# Autodesk Inventor assembly: Motor Panel
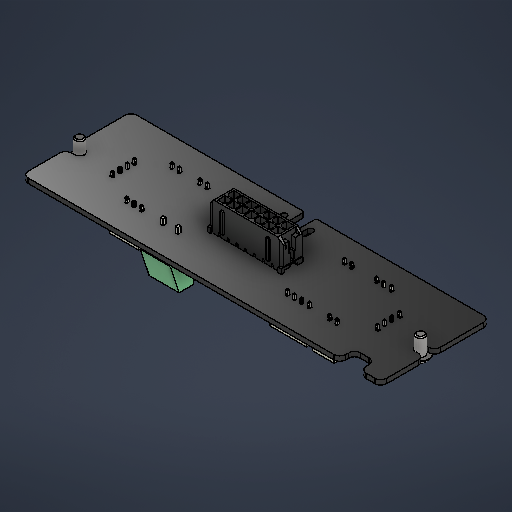
[picture p0: Inventor's stored thumbnail of the model, 512x512]
Saved by Autodesk Inventor 2026.1 (Build 301233020, 233B)
## iProperties
Created: 2025-05-09
Part Number: Motor Panel
Document SubType Name: Assembly
Designer: AdminForWorker
Title: Motor Panel
Author: AdminForWorker
## Documents named in this file (8)
- C:\Users\JoshuaEah\Documents\GitHub\Voron-0\CAD\Master Assembly\Panels\Subassemblies\Motor Panel.iam
- C:\Users\JoshuaEah\Documents\GitHub\Voron-0\CAD\Master Assembly\Hardware\M3x6 BHCS.ipt
- C:\Users\JoshuaEah\Documents\GitHub\Voron-0\CAD\Master Assembly\Electronics\Parts\Frame PCB.ipt
- C:\Users\JoshuaEah\Documents\GitHub\Voron-0\CAD\Master Assembly\Electronics\Parts\JST XH 2 Pin Female.ipt
- C:\Users\JoshuaEah\Documents\GitHub\Voron-0\CAD\Master Assembly\Electronics\Parts\JST XH 3 Pin Female.ipt
- C:\Users\JoshuaEah\Documents\GitHub\Voron-0\CAD\Master Assembly\Electronics\Parts\JST XH 4 Pin Female.ipt
- C:\Users\JoshuaEah\Documents\GitHub\Voron-0\CAD\Master Assembly\Electronics\Parts\Screw Terminal.ipt
- C:\Users\JoshuaEah\Documents\GitHub\Voron-0\CAD\Master Assembly\Electronics\Parts\Molex 14 Pin Female Straight.ipt
## Components (15 placed, 7 different names)
1. M3x6 BHCS:1
2. M3x6 BHCS:2
3. Frame PCB
4. JST XH 2 Pin Female:1
5. JST XH 2 Pin Female:2
6. JST XH 2 Pin Female:3
7. JST XH 2 Pin Female:4
8. JST XH 2 Pin Female:5
9. JST XH 3 Pin Female:1
10. JST XH 3 Pin Female:2
11. JST XH 4 Pin Female:1
12. JST XH 4 Pin Female:2
13. JST XH 4 Pin Female:3
14. Screw Terminal:1
15. Molex 14 Pin:1
## Relationships (3: Mate 3)
- [Mate]: M3x6 BHCS:1 ↔ Frame PCB
- [Mate]: M3x6 BHCS:2 ↔ Frame PCB
- [Mate]: M3x6 BHCS:1 ↔ Frame PCB
